# Autodesk Inventor assembly: main_assembly
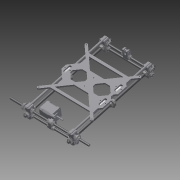
[picture p0: Inventor's stored thumbnail of the model, 180x180]
Saved by Autodesk Inventor 2015 (Build 190159000, 159)
## iProperties
Created: 2015-05-09
Part Number: main_assembly
Document SubType Name: Assembly
Designer: X
Author: X
## Documents named in this file (6)
- G:\3d printer\Prusa i3\CAD\main_assembly.iam
- G:\3d printer\Prusa i3\CAD\frame\platform_redrawn.ipt
- G:\3d printer\Prusa i3\CAD\3d_printer_part\y-belt-holder.ipt
- G:\3d printer\Prusa i3\CAD\chassis.iam
- G:\3d printer\Prusa i3\CAD\standard_parts\Imported Components\NEMA 17 Stepper Motor Assembly\NEMA 17 Stepper Motor Assembly.iam
- G:\3d printer\Prusa i3\CAD\standard_parts\LM8UU 8mm Linear Bearing.ipt
## Components (7 placed, 5 different names)
1. platform_redrawn:1 — Cylindrical:1, Cylindrical:2, Mate:1, Angle:1, Mate:3, Tangent:1, Tangent:2, Mate:4, Mate:5
2. y-belt-holder:1 — Cylindrical:1, Cylindrical:2, Mate:1
3. chassis:1 [sub-assembly] — Cylindrical:3, Cylindrical:4, Mate:2, Cylindrical:5, Cylindrical:6, Cylindrical:7, Angle:1
4. NEMA 17 Stepper Motor Assembly:1 [sub-assembly] — Cylindrical:3, Cylindrical:4, Mate:2
5. LM8UU 8mm Linear Bearing:1 — Cylindrical:6, Mate:3, Tangent:1, Tangent:2
6. LM8UU 8mm Linear Bearing:2 — Cylindrical:5, Mate:4
7. LM8UU 8mm Linear Bearing:3 — Cylindrical:7, Mate:5
## Relationships (15: CylindricalJoint 7, Mate 5, Tangent 2, Angle 1)
- Cylindrical:1: platform_redrawn:1 ↔ y-belt-holder:1
- Cylindrical:2: platform_redrawn:1 ↔ y-belt-holder:1
- Mate:1: platform_redrawn:1 ↔ y-belt-holder:1
- Cylindrical:3: chassis:1 ↔ NEMA 17 Stepper Motor Assembly:1
- Cylindrical:4: chassis:1 ↔ NEMA 17 Stepper Motor Assembly:1
- Mate:2: chassis:1 ↔ NEMA 17 Stepper Motor Assembly:1
- Cylindrical:5: chassis:1 ↔ LM8UU 8mm Linear Bearing:2
- Cylindrical:6: chassis:1 ↔ LM8UU 8mm Linear Bearing:1
- Cylindrical:7: chassis:1 ↔ LM8UU 8mm Linear Bearing:3
- Angle:1 (0 deg): platform_redrawn:1 ↔ chassis:1
- Mate:3 (3.5 mm): platform_redrawn:1 ↔ LM8UU 8mm Linear Bearing:1
- Tangent:1: platform_redrawn:1 ↔ LM8UU 8mm Linear Bearing:1
- Tangent:2: platform_redrawn:1 ↔ LM8UU 8mm Linear Bearing:1
- Mate:4 (3.5 mm): platform_redrawn:1 ↔ LM8UU 8mm Linear Bearing:2
- Mate:5 (3.5 mm): platform_redrawn:1 ↔ LM8UU 8mm Linear Bearing:3
